# Autodesk Inventor assembly: 203.004.01_ZB_Extrudereinheit
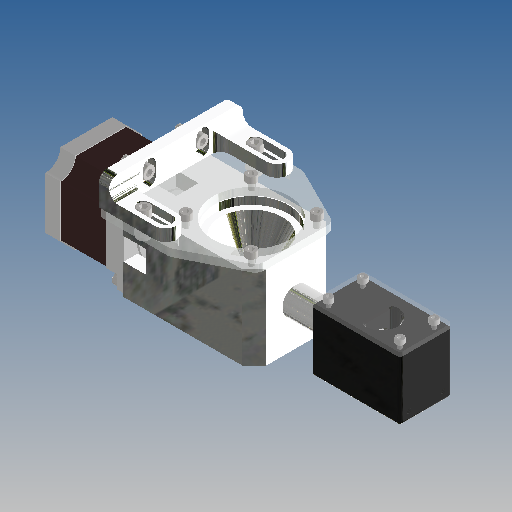
[picture p0: Inventor's stored thumbnail of the model, 512x512]
Saved by Autodesk Inventor 2021 (Build 250183000, 183)
## iProperties
Created: 2021-11-03
Part Number: 203.004.01_ZB_Extrudereinheit
Document SubType Name: Assembly
Designer: Sebastian Seewald
Author: Sebastian Seewald
## Documents named in this file (11)
- \\u262868-sub23.your-storagebox.de@SSL\DavWWWRoot\Master_Projekt_SS_2021\Projektdaten\50_Modul_Vereinzelung\55_Konstruktion\104_Extrudereinheit\204.003.01_ZB_Extruder.iam
- \\u262868-sub23.your-storagebox.de@SSL\DavWWWRoot\Master_Projekt_SS_2021\Projektdaten\50_Modul_Vereinzelung\55_Konstruktion\104_Extrudereinheit\504.003.01_MC18_Motor.ipt
- \\u262868-sub23.your-storagebox.de@SSL\DavWWWRoot\Master_Projekt_SS_2021\Projektdaten\50_Modul_Vereinzelung\55_Konstruktion\104_Extrudereinheit\104.003.01_MC18_Gehaeuse.ipt
- \\u262868-sub23.your-storagebox.de@SSL\DavWWWRoot\Master_Projekt_SS_2021\Projektdaten\50_Modul_Vereinzelung\55_Konstruktion\104_Extrudereinheit\504.006.01_MC18_Extruderwelle.ipt
- \\u262868-sub23.your-storagebox.de@SSL\DavWWWRoot\Master_Projekt_SS_2021\Projektdaten\50_Modul_Vereinzelung\55_Konstruktion\104_Extrudereinheit\104.004.01_MC18_Zwischenrohr.ipt
- \\u262868-sub23.your-storagebox.de@SSL\DavWWWRoot\Master_Projekt_SS_2021\Projektdaten\50_Modul_Vereinzelung\55_Konstruktion\104_Extrudereinheit\Schrauben\DIN EN ISO 4762 - M4 x 10.ipt
- \\u262868-sub23.your-storagebox.de@SSL\DavWWWRoot\Master_Projekt_SS_2021\Projektdaten\50_Modul_Vereinzelung\55_Konstruktion\104_Extrudereinheit\104.005.01_Dosiereinheit_Rahmenaufnahme.ipt
- \\u262868-sub23.your-storagebox.de@SSL\DavWWWRoot\Master_Projekt_SS_2021\Projektdaten\50_Modul_Vereinzelung\55_Konstruktion\104_Extrudereinheit\104.006.01_Einstellwinkel.ipt
- \\u262868-sub23.your-storagebox.de@SSL\DavWWWRoot\Master_Projekt_SS_2021\Projektdaten\50_Modul_Vereinzelung\55_Konstruktion\104_Extrudereinheit\Schrauben\DIN EN ISO 4762 - M5 x 12.ipt
- \\u262868-sub23.your-storagebox.de@SSL\DavWWWRoot\Master_Projekt_SS_2021\Projektdaten\50_Modul_Vereinzelung\55_Konstruktion\104_Extrudereinheit\Schrauben\ISO 10511 - M5 x 05 Mutter.ipt
- \\u262868-sub23.your-storagebox.de@SSL\DavWWWRoot\Master_Projekt_SS_2021\Projektdaten\50_Modul_Vereinzelung\55_Konstruktion\104_Extrudereinheit\204.004.01_ZB_Geranulatvorfuehrung.iam
## Components (21 placed, 10 different names)
1. 504.003.01_MC18_Motor:1 — Passend:4, Passend:5, Passend:6, Winkel:1, Passend:7, Passend:8, Passend:9, Passend:10, Passend:11, Passend:12, Passend:13, Passend:14
2. 104.003.01_MC18_Gehaeuse:1 — Passend:1, Passend:2, Passend:3, Passend:4, Passend:5, Passend:6, Passend:15, Passend:16, Passend:17, Winkel:2
3. 504.006.01_MC18_Extruderwelle:1 — Passend:3, Winkel:1, Fluchtend:1
4. 104.004.01_MC18_Zwischenrohr:1 — Passend:1, Passend:2, Fluchtend:1, Passend:41, Passend:48
5. DIN EN ISO 4762 - M4 x 10:1 — Passend:8, Passend:12
6. DIN EN ISO 4762 - M4 x 10:2 — Passend:7, Passend:13
7. DIN EN ISO 4762 - M4 x 10:3 — Passend:9, Passend:14
8. DIN EN ISO 4762 - M4 x 10:4 — Passend:10, Passend:11
9. 104.005.01_Dosiereinheit_Rahmenaufnahme:1 — Passend:15, Passend:16, Passend:17, Passend:18, Passend:19, Passend:20, Passend:21, Passend:22, Passend:23, Passend:24, Passend:25, Passend:26, Passend:36, Passend:37, Fluchtend:2, Fluchtend:3
10. DIN EN ISO 4762 - M4 x 10:5 — Passend:19, Passend:24
11. DIN EN ISO 4762 - M4 x 10:6 — Passend:18, Passend:23
12. DIN EN ISO 4762 - M4 x 10:7 — Passend:20, Passend:22
13. DIN EN ISO 4762 - M4 x 10:8 — Passend:21, Passend:25
14. 104.006.01_Einstellwinkel:1 — Passend:26, Passend:27, Passend:28, Fluchtend:2, Passend:38, Passend:39, Passend:42, Passend:43, Passend:44, Passend:45, Passend:46, Passend:47, Fluchtend:3
15. DIN EN ISO 4762 - M5 x 12:1 — Passend:27, Passend:34, Passend:38
16. DIN EN ISO 4762 - M5 x 12:2 — Passend:28, Passend:35, Passend:39
17. ISO 10511 - M5 x 05 Mutter:1 — Passend:34, Passend:36
18. ISO 10511 - M5 x 05 Mutter:2 — Passend:35, Passend:37
19. DIN EN ISO 4762 - M5 x 12:3 — Passend:42, Passend:45, Passend:46
20. DIN EN ISO 4762 - M5 x 12:4 — Passend:43, Passend:44, Passend:47
21. 204.004.01_ZB_Geranulatvorfuehrung:1 [sub-assembly] — Passend:41, Winkel:2, Passend:48
## Relationships (47: Mate 42, Flush 3, Angle 2)
- Passend:1 [Mate]: 104.003.01_MC18_Gehaeuse:1 ↔ 104.004.01_MC18_Zwischenrohr:1
- Passend:2 [Mate]: 104.003.01_MC18_Gehaeuse:1 ↔ 104.004.01_MC18_Zwischenrohr:1
- Passend:3 [Mate]: 104.003.01_MC18_Gehaeuse:1 ↔ 504.006.01_MC18_Extruderwelle:1
- Passend:4 [Mate]: 504.003.01_MC18_Motor:1 ↔ 104.003.01_MC18_Gehaeuse:1
- Passend:5 [Mate]: 504.003.01_MC18_Motor:1 ↔ 104.003.01_MC18_Gehaeuse:1
- Passend:6 [Mate]: 504.003.01_MC18_Motor:1 ↔ 104.003.01_MC18_Gehaeuse:1
- Winkel:1 [Angle] (0 deg): 504.003.01_MC18_Motor:1 ↔ 504.006.01_MC18_Extruderwelle:1
- Fluchtend:1 [Flush]: 504.006.01_MC18_Extruderwelle:1 ↔ 104.004.01_MC18_Zwischenrohr:1
- Passend:7 [Mate]: 504.003.01_MC18_Motor:1 ↔ DIN EN ISO 4762 - M4 x 10:2
- Passend:8 [Mate]: 504.003.01_MC18_Motor:1 ↔ DIN EN ISO 4762 - M4 x 10:1
- Passend:9 [Mate]: 504.003.01_MC18_Motor:1 ↔ DIN EN ISO 4762 - M4 x 10:3
- Passend:10 [Mate]: 504.003.01_MC18_Motor:1 ↔ DIN EN ISO 4762 - M4 x 10:4
- Passend:11 [Mate]: 504.003.01_MC18_Motor:1 ↔ DIN EN ISO 4762 - M4 x 10:4
- Passend:12 [Mate]: 504.003.01_MC18_Motor:1 ↔ DIN EN ISO 4762 - M4 x 10:1
- Passend:13 [Mate]: 504.003.01_MC18_Motor:1 ↔ DIN EN ISO 4762 - M4 x 10:2
- Passend:14 [Mate]: 504.003.01_MC18_Motor:1 ↔ DIN EN ISO 4762 - M4 x 10:3
- Passend:15 [Mate]: 104.003.01_MC18_Gehaeuse:1 ↔ 104.005.01_Dosiereinheit_Rahmenaufnahme:1
- Passend:16 [Mate]: 104.003.01_MC18_Gehaeuse:1 ↔ 104.005.01_Dosiereinheit_Rahmenaufnahme:1
- Passend:17 [Mate]: 104.003.01_MC18_Gehaeuse:1 ↔ 104.005.01_Dosiereinheit_Rahmenaufnahme:1
- Passend:18 [Mate]: 104.005.01_Dosiereinheit_Rahmenaufnahme:1 ↔ DIN EN ISO 4762 - M4 x 10:6
- Passend:19 [Mate]: 104.005.01_Dosiereinheit_Rahmenaufnahme:1 ↔ DIN EN ISO 4762 - M4 x 10:5
- Passend:20 [Mate]: 104.005.01_Dosiereinheit_Rahmenaufnahme:1 ↔ DIN EN ISO 4762 - M4 x 10:7
- Passend:21 [Mate]: 104.005.01_Dosiereinheit_Rahmenaufnahme:1 ↔ DIN EN ISO 4762 - M4 x 10:8
- Passend:22 [Mate]: 104.005.01_Dosiereinheit_Rahmenaufnahme:1 ↔ DIN EN ISO 4762 - M4 x 10:7
- Passend:23 [Mate]: 104.005.01_Dosiereinheit_Rahmenaufnahme:1 ↔ DIN EN ISO 4762 - M4 x 10:6
- Passend:24 [Mate]: 104.005.01_Dosiereinheit_Rahmenaufnahme:1 ↔ DIN EN ISO 4762 - M4 x 10:5
- Passend:25 [Mate]: 104.005.01_Dosiereinheit_Rahmenaufnahme:1 ↔ DIN EN ISO 4762 - M4 x 10:8
- Passend:26 [Mate]: 104.005.01_Dosiereinheit_Rahmenaufnahme:1 ↔ 104.006.01_Einstellwinkel:1
- Passend:27 [Mate]: 104.006.01_Einstellwinkel:1 ↔ DIN EN ISO 4762 - M5 x 12:1
- Passend:28 [Mate]: 104.006.01_Einstellwinkel:1 ↔ DIN EN ISO 4762 - M5 x 12:2
- Passend:34 [Mate]: DIN EN ISO 4762 - M5 x 12:1 ↔ ISO 10511 - M5 x 05 Mutter:1
- Passend:35 [Mate]: DIN EN ISO 4762 - M5 x 12:2 ↔ ISO 10511 - M5 x 05 Mutter:2
- Passend:36 [Mate]: 104.005.01_Dosiereinheit_Rahmenaufnahme:1 ↔ ISO 10511 - M5 x 05 Mutter:1
- Passend:37 [Mate]: 104.005.01_Dosiereinheit_Rahmenaufnahme:1 ↔ ISO 10511 - M5 x 05 Mutter:2
- Fluchtend:2 [Flush]: 104.005.01_Dosiereinheit_Rahmenaufnahme:1 ↔ 104.006.01_Einstellwinkel:1
- Passend:38 [Mate]: 104.006.01_Einstellwinkel:1 ↔ DIN EN ISO 4762 - M5 x 12:1
- Passend:39 [Mate]: 104.006.01_Einstellwinkel:1 ↔ DIN EN ISO 4762 - M5 x 12:2
- Passend:41 [Mate] (-27.5 mm): 104.004.01_MC18_Zwischenrohr:1 ↔ 204.004.01_ZB_Geranulatvorfuehrung:1
- Passend:42 [Mate]: 104.006.01_Einstellwinkel:1 ↔ DIN EN ISO 4762 - M5 x 12:3
- Passend:43 [Mate]: 104.006.01_Einstellwinkel:1 ↔ DIN EN ISO 4762 - M5 x 12:4
- Passend:44 [Mate] (2.6 mm): 104.006.01_Einstellwinkel:1 ↔ DIN EN ISO 4762 - M5 x 12:4
- Passend:45 [Mate] (2.6 mm): 104.006.01_Einstellwinkel:1 ↔ DIN EN ISO 4762 - M5 x 12:3
- Passend:46 [Mate] (4 mm): 104.006.01_Einstellwinkel:1 ↔ DIN EN ISO 4762 - M5 x 12:3
- Passend:47 [Mate] (4 mm): 104.006.01_Einstellwinkel:1 ↔ DIN EN ISO 4762 - M5 x 12:4
- Winkel:2 [Angle] (0 deg): 104.003.01_MC18_Gehaeuse:1 ↔ 204.004.01_ZB_Geranulatvorfuehrung:1
- Fluchtend:3 [Flush]: 104.005.01_Dosiereinheit_Rahmenaufnahme:1 ↔ 104.006.01_Einstellwinkel:1
- Passend:48 [Mate]: 104.004.01_MC18_Zwischenrohr:1 ↔ 204.004.01_ZB_Geranulatvorfuehrung:1
